# Autodesk Inventor assembly: Drivebase AM14U4 Square 28inx28in v411
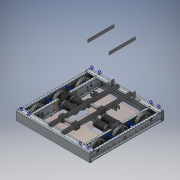
[picture p0: Inventor's stored thumbnail of the model, 180x180]
Saved by Autodesk Inventor 2018 (Build 220112000, 112)
## iProperties
Created: 2020-01-28
Part Number: Drivebase AM14U4 Square 28inx28in v411
Document SubType Name: Assembly
Designer: Weeb No1
Sending System: Autodesk Translation Framework v8.12.0.6
Preprocessor: ST-DEVELOPER v18
Title: /Users/GabG/Documents/GitHub/2020CAD/New Gabriel Shooter/Drivebase AM14U4 Square 28inx28in v41.step
## Documents named in this file (14)
- C:\Users\T3500STATIC\Documents\GitHub\2020CAD\Gabriel Inventor Files (Shooter, Drivebase)\Drivebase Assembly\Main Assembly\Drivebase AM14U4 Square 28inx28in v411.iam
- C:\Users\T3500STATIC\Documents\GitHub\2020CAD\Gabriel Inventor Files (Shooter, Drivebase)\Drivebase Assembly\Part Files\AM14U4 Square Half.iam
- C:\Users\T3500STATIC\Documents\GitHub\2020CAD\Gabriel Inventor Files (Shooter, Drivebase)\Drivebase Assembly\Part Files\AM14U4 Square Half_1.iam
- C:\Users\T3500STATIC\Documents\GitHub\2020CAD\Gabriel Inventor Files (Shooter, Drivebase)\Drivebase Assembly\Part Files\Placeholder Belly Pan.ipt
- C:\Users\T3500STATIC\Documents\GitHub\2020CAD\Gabriel Inventor Files (Shooter, Drivebase)\Drivebase Assembly\Part Files\10-24 Washer.ipt
- C:\Users\T3500STATIC\Documents\GitHub\2020CAD\Gabriel Inventor Files (Shooter, Drivebase)\Drivebase Assembly\Part Files\Bumper Assembly.iam
- C:\Users\T3500STATIC\Documents\GitHub\2020CAD\Gabriel Inventor Files (Shooter, Drivebase)\Drivebase Assembly\Part Files\Bumper Assembly_1.iam
- C:\Users\T3500STATIC\Documents\GitHub\2020CAD\Gabriel Inventor Files (Shooter, Drivebase)\Drivebase Assembly\Part Files\95335A503_METRIC QUICK-RELEASE PIN.ipt
- C:\Users\T3500STATIC\Documents\GitHub\2020CAD\Gabriel Inventor Files (Shooter, Drivebase)\Drivebase Assembly\Part Files\8020 1010 x 26 v2.ipt
- C:\Users\T3500STATIC\Documents\GitHub\2020CAD\Gabriel Inventor Files (Shooter, Drivebase)\Drivebase Assembly\Part Files\Component52.ipt
- C:\Users\T3500STATIC\Documents\GitHub\2020CAD\Tyler's Ball Storage\Polycarb half main conv.iam
- C:\Users\T3500STATIC\Documents\GitHub\2020CAD\Gabriel Inventor Files (Shooter, Drivebase)\Gussets\2in 4-hole Bracket 0.25in Hole.ipt
- C:\Users\T3500STATIC\Documents\GitHub\2020CAD\Gabriel Inventor Files (Shooter, Drivebase)\Shooter Curve Assembly\Part Files\8020 1010 x 1 5.ipt
- C:\Users\T3500STATIC\Documents\GitHub\2020CAD\Gabriel Inventor Files (Shooter, Drivebase)\Shooter Curve Assembly\Part Files\0.125 in Flatbar Support Beam.ipt
## Components (42 placed, 13 different names)
1. AM14U4 Square Half:1 [sub-assembly] — Mate:69, Mate:70, Mate:71, Mate:75, Mate:76, Mate:77, Mate:82, Mate:83, Mate:84, Mate:85, Mate:91, Mate:92, Mate:96, Mate:97, Symmetry:1, Mate:111, Mate:112, Mate:115, Mate:116, Mate:117, Mate:121, Mate:122, Mate:123, Mate:124, Mate:125
2. AM14U4 Square Half_1:1 [sub-assembly] — Mate:66, Mate:67, Mate:68, Mate:72, Mate:73, Mate:74, Mate:78, Mate:79, Mate:80, Mate:81, Mate:93, Mate:94, Mate:95, Mate:98, Symmetry:1, Mate:109, Mate:110, Mate:113, Mate:114
3. Placeholder Belly Pan:1 — Mate:91, Mate:92, Mate:93, Mate:94, Mate:95, Mate:96, Mate:97, Mate:98, Mate:99, Mate:100, Mate:101, Mate:102, Mate:103, Mate:104, Mate:105, Mate:106
4. 10-24 Washer:1 — Mate:101
5. 10-24 Washer:2 — Mate:102
6. 10-24 Washer:3 — Mate:100
7. 10-24 Washer:4 — Mate:99
8. 10-24 Washer:5 — Mate:106
9. 10-24 Washer:6 — Mate:105
10. 10-24 Washer:7 — Mate:104
11. 10-24 Washer:8 — Mate:103
12. Bumper Assembly:1 [sub-assembly] — Mate:72, Mate:73, Mate:74, Mate:75, Mate:76, Mate:77
13. Bumper Assembly_1:1 [sub-assembly] — Mate:66, Mate:67, Mate:68, Mate:69, Mate:70, Mate:71
14. 95335A503_METRIC QUICK-RELEASE PIN:1 — Mate:82
15. 95335A503_METRIC QUICK-RELEASE PIN:2 — Mate:83
16. 95335A503_METRIC QUICK-RELEASE PIN:3 — Mate:85
17. 95335A503_METRIC QUICK-RELEASE PIN:4 — Mate:84
18. 95335A503_METRIC QUICK-RELEASE PIN:5 — Mate:78
19. 95335A503_METRIC QUICK-RELEASE PIN:6 — Mate:79
20. 95335A503_METRIC QUICK-RELEASE PIN:7 — Mate:80
21. 95335A503_METRIC QUICK-RELEASE PIN:8 — Mate:81
22. 8020 1010 x 26 v2:1 — Mate:107, Mate:113, Mate:114, Mate:115, Mate:116, Flush:3, Mate:130, Mate:132, Flush:6, Mate:137, Flush:17, Flush:18, Mate:140, Flush:19, Flush:20, Mate:142, Flush:21, Flush:22, Mate:144, Flush:23, Flush:24, Mate:151, Mate:152, Mate:153, Mate:154
23. 8020 1010 x 26 v2:2 — Mate:108, Mate:109, Mate:110, Mate:111, Mate:112, Mate:133, Flush:9, Mate:134, Flush:12, Mate:136, Flush:15, Flush:16, Mate:145, Flush:25, Flush:26, Mate:147, Flush:27, Flush:28, Mate:149, Flush:29, Flush:30
24. Component52:1
25. Polycarb half main conv:1 [sub-assembly] — Mate:151, Mate:152
26. Polycarb half main conv:3 [sub-assembly] — Mate:153, Mate:154
27. 2in 4-hole Bracket 0.25in Hole:1 — Mate:121, Mate:122, Mate:123
28. 2in 4-hole Bracket 0.25in Hole:2 — Mate:117, Mate:124, Mate:125
29. 8020 1010 x 1 5:1 — Flush:3, Mate:130
30. 8020 1010 x 1 5:2 — Mate:134, Flush:12
31. 8020 1010 x 1 5:3 — Mate:133, Flush:9
32. 8020 1010 x 1 5:4 — Mate:132, Flush:6
33. 2in 4-hole Bracket 0.25in Hole:3 — Mate:137, Flush:17, Flush:18
34. 2in 4-hole Bracket 0.25in Hole:4 — Mate:136, Flush:15, Flush:16
35. 2in 4-hole Bracket 0.25in Hole:5 — Mate:149, Flush:29, Flush:30
36. 2in 4-hole Bracket 0.25in Hole:6 — Mate:144, Flush:23, Flush:24
37. 2in 4-hole Bracket 0.25in Hole:7 — Mate:140, Flush:19, Flush:20
38. 2in 4-hole Bracket 0.25in Hole:8 — Mate:142, Flush:21, Flush:22
39. 2in 4-hole Bracket 0.25in Hole:9 — Mate:147, Flush:27, Flush:28
40. 2in 4-hole Bracket 0.25in Hole:10 — Mate:145, Flush:25, Flush:26
41. 0.125 in Flatbar Support Beam:1
42. 0.125 in Flatbar Support Beam:2
## Relationships (89: Mate 68, Flush 20, Symmetry 1)
- Mate:66: AM14U4 Square Half_1:1 ↔ Bumper Assembly_1:1
- Mate:67: AM14U4 Square Half_1:1 ↔ Bumper Assembly_1:1
- Mate:68: AM14U4 Square Half_1:1 ↔ Bumper Assembly_1:1
- Mate:69: AM14U4 Square Half:1 ↔ Bumper Assembly_1:1
- Mate:70: AM14U4 Square Half:1 ↔ Bumper Assembly_1:1
- Mate:71: AM14U4 Square Half:1 ↔ Bumper Assembly_1:1
- Mate:72: AM14U4 Square Half_1:1 ↔ Bumper Assembly:1
- Mate:73: AM14U4 Square Half_1:1 ↔ Bumper Assembly:1
- Mate:74: AM14U4 Square Half_1:1 ↔ Bumper Assembly:1
- Mate:75: AM14U4 Square Half:1 ↔ Bumper Assembly:1
- Mate:76: AM14U4 Square Half:1 ↔ Bumper Assembly:1
- Mate:77: AM14U4 Square Half:1 ↔ Bumper Assembly:1
- Mate:78: AM14U4 Square Half_1:1 ↔ 95335A503_METRIC QUICK-RELEASE PIN:5
- Mate:79: AM14U4 Square Half_1:1 ↔ 95335A503_METRIC QUICK-RELEASE PIN:6
- Mate:80: AM14U4 Square Half_1:1 ↔ 95335A503_METRIC QUICK-RELEASE PIN:7
- Mate:81: AM14U4 Square Half_1:1 ↔ 95335A503_METRIC QUICK-RELEASE PIN:8
- Mate:82: AM14U4 Square Half:1 ↔ 95335A503_METRIC QUICK-RELEASE PIN:1
- Mate:83: AM14U4 Square Half:1 ↔ 95335A503_METRIC QUICK-RELEASE PIN:2
- Mate:84: AM14U4 Square Half:1 ↔ 95335A503_METRIC QUICK-RELEASE PIN:4
- Mate:85: AM14U4 Square Half:1 ↔ 95335A503_METRIC QUICK-RELEASE PIN:3
- Mate:91: AM14U4 Square Half:1 ↔ Placeholder Belly Pan:1
- Mate:92: AM14U4 Square Half:1 ↔ Placeholder Belly Pan:1
- Mate:93: AM14U4 Square Half_1:1 ↔ Placeholder Belly Pan:1
- Mate:94: AM14U4 Square Half_1:1 ↔ Placeholder Belly Pan:1
- Mate:95: AM14U4 Square Half_1:1 ↔ Placeholder Belly Pan:1
- Mate:96: AM14U4 Square Half:1 ↔ Placeholder Belly Pan:1
- Mate:97: AM14U4 Square Half:1 ↔ Placeholder Belly Pan:1
- Mate:98: AM14U4 Square Half_1:1 ↔ Placeholder Belly Pan:1
- Mate:99: Placeholder Belly Pan:1 ↔ 10-24 Washer:4
- Mate:100: Placeholder Belly Pan:1 ↔ 10-24 Washer:3
- Mate:101: Placeholder Belly Pan:1 ↔ 10-24 Washer:1
- Mate:102: Placeholder Belly Pan:1 ↔ 10-24 Washer:2
- Mate:103: Placeholder Belly Pan:1 ↔ 10-24 Washer:8
- Mate:104: Placeholder Belly Pan:1 ↔ 10-24 Washer:7
- Mate:105: Placeholder Belly Pan:1 ↔ 10-24 Washer:6
- Mate:106: Placeholder Belly Pan:1 ↔ 10-24 Washer:5
- Symmetry:1: AM14U4 Square Half:1 ↔ AM14U4 Square Half_1:1
- Mate:107 (57.15 mm): 8020 1010 x 26 v2:1
- Mate:108 (-69.85 mm): 8020 1010 x 26 v2:2
- Mate:109 (-25.019 mm): AM14U4 Square Half_1:1 ↔ 8020 1010 x 26 v2:2
- Mate:110: AM14U4 Square Half_1:1 ↔ 8020 1010 x 26 v2:2
- Mate:111: AM14U4 Square Half:1 ↔ 8020 1010 x 26 v2:2
- Mate:112 (-24.257 mm): AM14U4 Square Half:1 ↔ 8020 1010 x 26 v2:2
- Mate:113 (-25.019 mm): AM14U4 Square Half_1:1 ↔ 8020 1010 x 26 v2:1
- Mate:114: AM14U4 Square Half_1:1 ↔ 8020 1010 x 26 v2:1
- Mate:115: AM14U4 Square Half:1 ↔ 8020 1010 x 26 v2:1
- Mate:116 (-24.257 mm): AM14U4 Square Half:1 ↔ 8020 1010 x 26 v2:1
- Mate:117: AM14U4 Square Half:1 ↔ 2in 4-hole Bracket 0.25in Hole:2
- Mate:121: AM14U4 Square Half:1 ↔ 2in 4-hole Bracket 0.25in Hole:1
- Mate:122: AM14U4 Square Half:1 ↔ 2in 4-hole Bracket 0.25in Hole:1
- Mate:123: AM14U4 Square Half:1 ↔ 2in 4-hole Bracket 0.25in Hole:1
- Mate:124: AM14U4 Square Half:1 ↔ 2in 4-hole Bracket 0.25in Hole:2
- Mate:125: AM14U4 Square Half:1 ↔ 2in 4-hole Bracket 0.25in Hole:2
- Flush:3: 8020 1010 x 26 v2:1 ↔ 8020 1010 x 1 5:1
- Mate:130: 8020 1010 x 26 v2:1 ↔ 8020 1010 x 1 5:1
- Mate:132: 8020 1010 x 26 v2:1 ↔ 8020 1010 x 1 5:4
- Flush:6: 8020 1010 x 26 v2:1 ↔ 8020 1010 x 1 5:4
- Mate:133: 8020 1010 x 26 v2:2 ↔ 8020 1010 x 1 5:3
- Flush:9: 8020 1010 x 26 v2:2 ↔ 8020 1010 x 1 5:3
- Mate:134: 8020 1010 x 26 v2:2 ↔ 8020 1010 x 1 5:2
- Flush:12: 8020 1010 x 26 v2:2 ↔ 8020 1010 x 1 5:2
- Mate:136: 8020 1010 x 26 v2:2 ↔ 2in 4-hole Bracket 0.25in Hole:4
- Flush:15: 8020 1010 x 26 v2:2 ↔ 2in 4-hole Bracket 0.25in Hole:4
- Flush:16: 8020 1010 x 26 v2:2 ↔ 2in 4-hole Bracket 0.25in Hole:4
- Mate:137: 8020 1010 x 26 v2:1 ↔ 2in 4-hole Bracket 0.25in Hole:3
- Flush:17: 8020 1010 x 26 v2:1 ↔ 2in 4-hole Bracket 0.25in Hole:3
- Flush:18: 8020 1010 x 26 v2:1 ↔ 2in 4-hole Bracket 0.25in Hole:3
- Mate:140: 8020 1010 x 26 v2:1 ↔ 2in 4-hole Bracket 0.25in Hole:7
- Flush:19: 8020 1010 x 26 v2:1 ↔ 2in 4-hole Bracket 0.25in Hole:7
- Flush:20: 8020 1010 x 26 v2:1 ↔ 2in 4-hole Bracket 0.25in Hole:7
- Mate:142: 8020 1010 x 26 v2:1 ↔ 2in 4-hole Bracket 0.25in Hole:8
- Flush:21: 8020 1010 x 26 v2:1 ↔ 2in 4-hole Bracket 0.25in Hole:8
- Flush:22: 8020 1010 x 26 v2:1 ↔ 2in 4-hole Bracket 0.25in Hole:8
- Mate:144: 8020 1010 x 26 v2:1 ↔ 2in 4-hole Bracket 0.25in Hole:6
- Flush:23: 8020 1010 x 26 v2:1 ↔ 2in 4-hole Bracket 0.25in Hole:6
- Flush:24: 8020 1010 x 26 v2:1 ↔ 2in 4-hole Bracket 0.25in Hole:6
- Mate:145: 8020 1010 x 26 v2:2 ↔ 2in 4-hole Bracket 0.25in Hole:10
- Flush:25: 8020 1010 x 26 v2:2 ↔ 2in 4-hole Bracket 0.25in Hole:10
- Flush:26: 8020 1010 x 26 v2:2 ↔ 2in 4-hole Bracket 0.25in Hole:10
- Mate:147: 8020 1010 x 26 v2:2 ↔ 2in 4-hole Bracket 0.25in Hole:9
- Flush:27: 8020 1010 x 26 v2:2 ↔ 2in 4-hole Bracket 0.25in Hole:9
- Flush:28: 8020 1010 x 26 v2:2 ↔ 2in 4-hole Bracket 0.25in Hole:9
- Mate:149: 8020 1010 x 26 v2:2 ↔ 2in 4-hole Bracket 0.25in Hole:5
- Flush:29: 8020 1010 x 26 v2:2 ↔ 2in 4-hole Bracket 0.25in Hole:5
- Flush:30: 8020 1010 x 26 v2:2 ↔ 2in 4-hole Bracket 0.25in Hole:5
- Mate:151: 8020 1010 x 26 v2:1 ↔ Polycarb half main conv:1
- Mate:152: 8020 1010 x 26 v2:1 ↔ Polycarb half main conv:1
- Mate:153: 8020 1010 x 26 v2:1 ↔ Polycarb half main conv:3
- Mate:154: 8020 1010 x 26 v2:1 ↔ Polycarb half main conv:3
